# Autodesk Inventor assembly: ASM0001_ASM
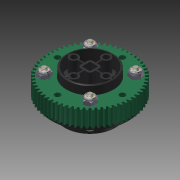
[picture p0: Inventor's stored thumbnail of the model, 180x180]
Saved by Autodesk Inventor 2015 SP1 (Build 190201100, 201)
## iProperties
Created: 2011-04-20
Part Number: ASM0001_ASM
Document SubType Name: Assembly
Designer: Jordan
Mass: 52.8067 g
Surface Area: 451.564 cm^2
Volume: 34.6205 cm^3
Density: 1.5253 g/cm^3
Author: Jordan
## Documents named in this file (7)
- C:\Users\Jordan\Documents\Robotics\VEX\CAD\2015 BNS CAD Library (beta)\Motion\Advanced Gears\60-Tooth Turntable Bearing.iam
- C:\Users\Jordan\Documents\Robotics\VEX\CAD\2015 BNS CAD Library (beta)\Motion\Advanced Gears\Reference Parts\60-Tooth Turntable Bearing\Middle.ipt
- C:\Users\Jordan\Documents\Robotics\VEX\CAD\2015 BNS CAD Library (beta)\Motion\Advanced Gears\Reference Parts\60-Tooth Turntable Bearing\Top.ipt
- C:\Users\Jordan\Documents\Robotics\VEX\CAD\2015 BNS CAD Library (beta)\Motion\Advanced Gears\Reference Parts\60-Tooth Turntable Bearing\60-Tooth Spur Gear.ipt
- C:\Users\Jordan\Documents\Robotics\VEX\CAD\2015 BNS CAD Library (beta)\Motion\Advanced Gears\Reference Parts\60-Tooth Turntable Bearing\Bottom.ipt
- C:\Users\Jordan\Documents\Robotics\VEX\CAD\2015 BNS CAD Library (beta)\Structure\Screws & Nuts\Screw 8-32 x 0.875''.ipt
- C:\Users\Jordan\Documents\Robotics\VEX\CAD\2015 BNS CAD Library (beta)\Structure\Screws & Nuts\Nut 8-32 Nylock.ipt
## Components (12 placed, 6 different names)
1. Middle:1 — Mate:3, Mate:4, Mate:6, Mate:7, Mate:8
2. Nut 8-32 Nylock:5 — Mate:15, Mate:16
3. Top:1 — Mate:5, Mate:23, Mate:24
4. 60-Tooth Spur Gear:1 — Mate:6, Mate:7, Mate:8, Mate:15, Mate:17, Mate:19, Mate:21, Mate:23, Mate:24
5. Nut 8-32 Nylock:6 — Mate:21, Mate:22
6. Screw 8-32 x 0.875'':1 — Mate:1, Mate:2, Mate:16
7. Screw 8-32 x 0.875'':2 — Mate:13, Mate:14, Mate:22
8. Nut 8-32 Nylock:7 — Mate:19, Mate:20
9. Screw 8-32 x 0.875'':3 — Mate:9, Mate:10, Mate:18
10. Screw 8-32 x 0.875'':4 — Mate:11, Mate:12, Mate:20
11. Bottom:1 — Mate:1, Mate:2, Mate:3, Mate:4, Mate:5, Mate:9, Mate:10, Mate:11, Mate:12, Mate:13, Mate:14
12. Nut 8-32 Nylock:8 — Mate:17, Mate:18
## Relationships (24: Mate 24)
- Mate:1: Screw 8-32 x 0.875'':1 ↔ Bottom:1
- Mate:2: Screw 8-32 x 0.875'':1 ↔ Bottom:1
- Mate:3: Middle:1 ↔ Bottom:1
- Mate:4: Middle:1 ↔ Bottom:1
- Mate:5: Top:1 ↔ Bottom:1
- Mate:6: Middle:1 ↔ 60-Tooth Spur Gear:1
- Mate:7: Middle:1 ↔ 60-Tooth Spur Gear:1
- Mate:8: Middle:1 ↔ 60-Tooth Spur Gear:1
- Mate:9: Screw 8-32 x 0.875'':3 ↔ Bottom:1
- Mate:10: Screw 8-32 x 0.875'':3 ↔ Bottom:1
- Mate:11: Screw 8-32 x 0.875'':4 ↔ Bottom:1
- Mate:12: Screw 8-32 x 0.875'':4 ↔ Bottom:1
- Mate:13: Screw 8-32 x 0.875'':2 ↔ Bottom:1
- Mate:14: Screw 8-32 x 0.875'':2 ↔ Bottom:1
- Mate:15: Nut 8-32 Nylock:5 ↔ 60-Tooth Spur Gear:1
- Mate:16: Nut 8-32 Nylock:5 ↔ Screw 8-32 x 0.875'':1
- Mate:17: 60-Tooth Spur Gear:1 ↔ Nut 8-32 Nylock:8
- Mate:18: Screw 8-32 x 0.875'':3 ↔ Nut 8-32 Nylock:8
- Mate:19: 60-Tooth Spur Gear:1 ↔ Nut 8-32 Nylock:7
- Mate:20: Nut 8-32 Nylock:7 ↔ Screw 8-32 x 0.875'':4
- Mate:21: 60-Tooth Spur Gear:1 ↔ Nut 8-32 Nylock:6
- Mate:22: Nut 8-32 Nylock:6 ↔ Screw 8-32 x 0.875'':2
- Mate:23: Top:1 ↔ 60-Tooth Spur Gear:1
- Mate:24: Top:1 ↔ 60-Tooth Spur Gear:1
